# Autodesk Inventor assembly: fixed_robot
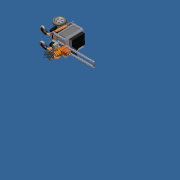
[picture p0: Inventor's stored thumbnail of the model, 180x180]
Saved by Autodesk Inventor 2012 (Build 160160000, 160)
## iProperties
Created: 2012-03-08
Part Number: fixed_robot
Document SubType Name: Assembly
Designer: esv
Mass: 186693 g
Surface Area: 125384 cm^2
Volume: 159546 cm^3
Density: 1.17015 g/cm^3
Author: esv
## Documents named in this file (7)
- C:\Users\Edward\Documents\masters\CAD\fixed_robot.iam
- C:\Users\Edward\Documents\masters\CAD\IRB120\IRB120.iam
- C:\Users\Edward\Documents\masters\CAD\Gripper\gripper.iam
- C:\Users\Edward\Documents\masters\CAD\Gripper\gripper jaw.iam
- C:\Users\Edward\Documents\masters\CAD\Invacare\caster assy.iam
- C:\Users\Edward\Documents\masters\CAD\Invacare\wheel.ipt
- C:\Users\Edward\Documents\masters\CAD\robot_solid.iam
## Components (9 placed, 6 different names)
1. caster assy:1 [sub-assembly] — Insert:3
2. wheel:1 — Insert:2
3. caster assy:2 [sub-assembly] — Insert:4
4. wheel:2 — Insert:1
5. robot_solid:1 [sub-assembly] — Insert:1, Insert:2, Insert:3, Insert:4, Tangent:1, Mate:57, Mate:58
6. IRB120:1 [sub-assembly] — Tangent:1, Mate:57, Mate:58, Insert:5, Insert:6
7. gripper:1 [sub-assembly] — Flush:43, Mate:60, Flush:44, Insert:5, Insert:6
8. gripper jaw:1 [sub-assembly] — Mate:59, Flush:41, Flush:42, Flush:43, Flush:44
9. gripper jaw:2 [sub-assembly] — Mate:59, Flush:41, Flush:42, Mate:60
## Relationships (17: Insert 6, Flush 5, Mate 5, Tangent 1)
- Flush:40 (-368.3 mm)
- Mate:56
- Insert:1: wheel:2 ↔ robot_solid:1
- Insert:2: wheel:1 ↔ robot_solid:1
- Insert:3: caster assy:1 ↔ robot_solid:1
- Insert:4: caster assy:2 ↔ robot_solid:1
- Tangent:1: robot_solid:1 ↔ IRB120:1
- Mate:57: robot_solid:1 ↔ IRB120:1
- Mate:58 (-508 mm): robot_solid:1 ↔ IRB120:1
- Mate:59 (50.8 mm): gripper jaw:1 ↔ gripper jaw:2
- Flush:41: gripper jaw:1 ↔ gripper jaw:2
- Flush:42: gripper jaw:1 ↔ gripper jaw:2
- Flush:43: gripper:1 ↔ gripper jaw:1
- Mate:60: gripper:1 ↔ gripper jaw:2
- Flush:44: gripper:1 ↔ gripper jaw:1
- Insert:5: IRB120:1 ↔ gripper:1
- Insert:6: IRB120:1 ↔ gripper:1
